# Autodesk Inventor assembly: Casserole
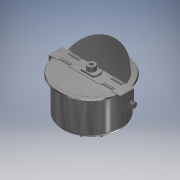
[picture p0: Inventor's stored thumbnail of the model, 180x180]
Saved by Autodesk Inventor 2017 (Build 210142000, 142)
## iProperties
Company: FABLAB Frenchmakers
Part Number: Casserole
Material: Générique
Document SubType Name: Assembly
Designer: FABLAB Frenchmakers
Mass: 4040.79 g
Surface Area: 1402.82 cm^2
Volume: 541.123 cm^3
Density: 7.46742 g/cm^3
Project: 1400-PopCorn Machine
Stock Number: 1400-01-00
Catalog Web Link: http://www.frenchmakers.com/
Author: Adrien MARY
## Documents named in this file (6)
- D:\Desktop\1400 Popcorn Machine\1400-01 Casserole\1400-01-00 Casserole.iam
- D:\Desktop\1400 Popcorn Machine\1400-01 Casserole\1400-01-01 Bol.ipt
- D:\Desktop\1400 Popcorn Machine\1400-01 Casserole\1400-01-03 Maintient_courvercle.ipt
- D:\Desktop\1400 Popcorn Machine\1400-01 Casserole\1400-01-02 Couvercle.ipt
- D:\Desktop\1400 Popcorn Machine\1400-01 Casserole\1400-01-08 Prise.ipt
- D:\Desktop\1400 Popcorn Machine\1400-01 Casserole\1400-01-07 Barre.ipt
## Components (6 placed, 5 different names)
1. 1400-01-01 Bol:1 — Affleurement:1, Affleurement:2, Affleurement:3, Placage:1, Angle:1, Angle:2, Placage:12, Placage:13, Placage:15
2. 1400-01-03 Maintient_courvercle:1 — Placage:1, Placage:2, Affleurement:4, Placage:10, Placage:11, Affleurement:16, Affleurement:17
3. 1400-01-02 Couvercle:1 — Affleurement:8, Affleurement:9, Placage:11, Angle:1
4. 1400-01-02 Couvercle:2 — Affleurement:9, Placage:10, Angle:2
5. 1400-01-08 Prise:1 — Placage:12, Placage:13, Angle:15
6. 1400-01-07 Barre:1 — Affleurement:16, Placage:15, Affleurement:17
## Relationships (18: Flush 8, Mate 7, Angle 3)
- Affleurement:1 [Flush]: 1400-01-01 Bol:1
- Affleurement:2 [Flush]: 1400-01-01 Bol:1
- Affleurement:3 [Flush]: 1400-01-01 Bol:1
- Placage:1 [Mate]: 1400-01-01 Bol:1 ↔ 1400-01-03 Maintient_courvercle:1
- Placage:2 [Mate]: 1400-01-03 Maintient_courvercle:1
- Affleurement:4 [Flush]: 1400-01-03 Maintient_courvercle:1
- Affleurement:8 [Flush]: 1400-01-02 Couvercle:1
- Affleurement:9 [Flush]: 1400-01-02 Couvercle:1 ↔ 1400-01-02 Couvercle:2
- Placage:10 [Mate]: 1400-01-03 Maintient_courvercle:1 ↔ 1400-01-02 Couvercle:2
- Placage:11 [Mate]: 1400-01-03 Maintient_courvercle:1 ↔ 1400-01-02 Couvercle:1
- Angle:1 (180 deg): 1400-01-01 Bol:1 ↔ 1400-01-02 Couvercle:1
- Angle:2 (137.5 deg): 1400-01-01 Bol:1 ↔ 1400-01-02 Couvercle:2
- Placage:12 [Mate]: 1400-01-01 Bol:1 ↔ 1400-01-08 Prise:1
- Placage:13 [Mate]: 1400-01-01 Bol:1 ↔ 1400-01-08 Prise:1
- Angle:15 (-45 deg): 1400-01-08 Prise:1
- Affleurement:16 [Flush]: 1400-01-03 Maintient_courvercle:1 ↔ 1400-01-07 Barre:1
- Placage:15 [Mate] (3 mm): 1400-01-01 Bol:1 ↔ 1400-01-07 Barre:1
- Affleurement:17 [Flush] (10 mm): 1400-01-03 Maintient_courvercle:1 ↔ 1400-01-07 Barre:1
## Named parameters: Ouverture = 42.5 deg
